# Autodesk Inventor assembly: New Detection Region
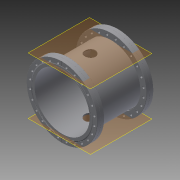
[picture p0: Inventor's stored thumbnail of the model, 180x180]
Saved by Autodesk Inventor 2014 (Build 180170000, 170)
## iProperties
Created: 2014-04-14
Part Number: New Detection Region
Document SubType Name: Assembly
Designer: ijs09
Author: Unknown
Title: Q:/STANDARDS/Web Drawings/Flanges/CF Flange/Flanges/10.00/Cleaned dxf/FN-1000.stp
Organization: Unknown
Description: Unknown
Sending System: Unknown
Preprocessor: XStep 1.0
Author: ijs09
## Documents named in this file (4)
- \\icnas3.cc.ic.ac.uk\ijs09\Inventor\New Detection Region.iam
- \\icnas3.cc.ic.ac.uk\ijs09\Inventor\P0000289.ipt
- \\icnas3.cc.ic.ac.uk\ijs09\Inventor\A0000684.iam
- \\icnas3.cc.ic.ac.uk\ijs09\Inventor\VacuumCylinder.ipt
## Components (3 placed, 3 different names)
1. P0000289 — Mate:1, Mate:2
2. A0000684 [sub-assembly] — Mate:3
3. VacuumCylinder:1 — Mate:1, Mate:2, Mate:3
## Relationships (3: Mate 3)
- Mate:1: P0000289 ↔ VacuumCylinder:1
- Mate:2: P0000289 ↔ VacuumCylinder:1
- Mate:3: A0000684 ↔ VacuumCylinder:1
